# Autodesk Inventor assembly: assembly
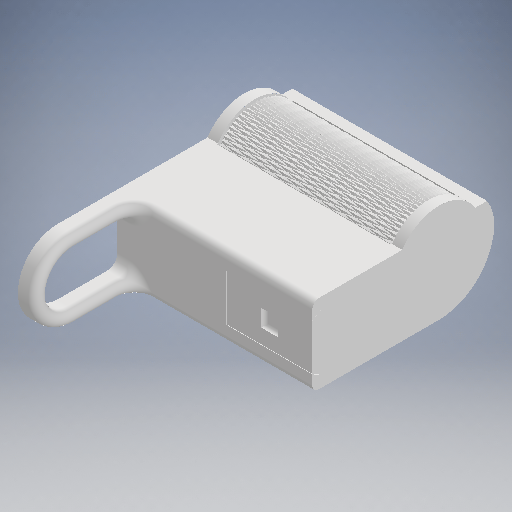
[picture p0: Inventor's stored thumbnail of the model, 512x512]
Saved by Autodesk Inventor 2025.2 (Build 292293000, 293)
## iProperties
Created: 2025-03-09
Part Number: assembly
Document SubType Name: Assembly
Designer: Alex
Author: Alex
## Documents named in this file (4)
- C:\Shared\alex-bartella-schoolwork\4b03\a1\a1.2\pack\assembly.iam
- C:\Shared\alex-bartella-schoolwork\4b03\a1\a1.2\pack\body.ipt
- C:\Shared\alex-bartella-schoolwork\4b03\a1\a1.2\pack\roller.ipt
- C:\Shared\alex-bartella-schoolwork\4b03\a1\a1.2\pack\door.ipt
## Components (3 placed, 3 different names)
1. body:1 — Mate:1, Mate:2, Mate:3, Mate:4, Mate:5, Mate:6, Flush:1
2. roller:1 — Mate:2, Mate:3, Mate:4
3. door:1 — Mate:5, Mate:6, Flush:1
## Relationships (7: Mate 6, Flush 1)
- Mate:1: body:1
- Mate:2: body:1 ↔ roller:1
- Mate:3 (0.3 mm): body:1 ↔ roller:1
- Mate:4: body:1 ↔ roller:1
- Mate:5 (0.1 mm): body:1 ↔ door:1
- Mate:6 (0.1 mm): body:1 ↔ door:1
- Flush:1: body:1 ↔ door:1
